# Autodesk Inventor assembly: ensamble 7-704
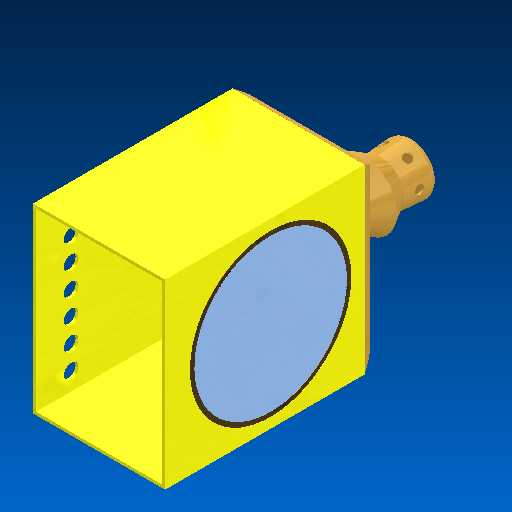
[picture p0: Inventor's stored thumbnail of the model, 512x512]
Saved by Autodesk Inventor 2025.2 (Build 292293000, 293)
## iProperties
Created: 2024-11-13
Part Number: ensamble 7-704
Document SubType Name: Assembly
Designer: Steven C
Author: Steven C
## Documents named in this file (6)
- C:\Users\Steven C\Desktop\ensamble7-704\ensamble 7-704.iam
- C:\Users\Steven C\Desktop\ensamble7-704\7-32.ipt
- C:\Users\Steven C\Desktop\ensamble7-704\Hudson-07-34.ipt
- C:\Users\Steven C\Desktop\ensamble7-704\Hudson-07-35-BASE.ipt
- C:\Users\Steven C\Desktop\ensamble7-704\Hudson-07-35-ESPEJO.ipt
- C:\Users\Steven C\Desktop\ensamble7-704\Hudson-07-36.ipt
## Components (5 placed, 5 different names)
1. 7-32:1 — De rotación:1, Coincidencia:1, Coincidencia:2, Coincidencia:3
2. Hudson-07-34:1 — De rotación:3
3. Hudson-07-35-BASE:1 — De rotación:1, De rotación:2, De rotación:3
4. Hudson-07-35-ESPEJO:1 — De rotación:2
5. Hudson-07-36:1 — Coincidencia:1, Coincidencia:2, Coincidencia:3
## Relationships (6: RevoluteJoint 3, Mate 3)
- De rotación:1 [RevoluteJoint]: 7-32:1 ↔ Hudson-07-35-BASE:1
- De rotación:2 [RevoluteJoint]: Hudson-07-35-BASE:1 ↔ Hudson-07-35-ESPEJO:1
- De rotación:3 [RevoluteJoint]: Hudson-07-34:1 ↔ Hudson-07-35-BASE:1
- Coincidencia:1 [Mate]: 7-32:1 ↔ Hudson-07-36:1
- Coincidencia:2 [Mate]: 7-32:1 ↔ Hudson-07-36:1
- Coincidencia:3 [Mate]: 7-32:1 ↔ Hudson-07-36:1
